# Autodesk Inventor assembly: Ensamble
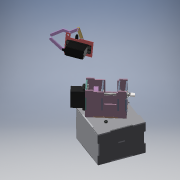
[picture p0: Inventor's stored thumbnail of the model, 180x180]
Saved by Autodesk Inventor 2019 (Build 230136000, 136)
## iProperties
Created: 2020-02-12
Part Number: Ensamble
Material: Genérico
Document SubType Name: Assembly
Designer: omar-
Author: omar-
## Documents named in this file (30)
- C:\Users\omar-\Documents\OMAR\BrazoRobotico\SERVOS\Diseño2\Ensamble.iam
- C:\Users\omar-\Documents\OMAR\BrazoRobotico\SERVOS\Diseño2\Piezas\BASE_FONDO.ipt
- C:\Users\omar-\Documents\OMAR\BrazoRobotico\SERVOS\Diseño2\Piezas\BASE_SOST.SERVO.ipt
- C:\Users\omar-\Documents\OMAR\BrazoRobotico\SERVOS\Diseño2\Servos\HS-322HD.ipt
- C:\Users\omar-\Documents\OMAR\BrazoRobotico\SERVOS\Diseño2\Piezas\BASE_TAPAFIJA.ipt
- C:\Users\omar-\Documents\OMAR\BrazoRobotico\SERVOS\Diseño2\Piezas\BASE_TAPA.ipt
- C:\Users\omar-\Documents\OMAR\BrazoRobotico\SERVOS\Diseño2\Piezas\BASE_TECHO.ipt
- C:\Users\omar-\Documents\OMAR\BrazoRobotico\SERVOS\Diseño2\Piezas\BASE_SOST.INFERIOR.ipt
- C:\Users\omar-\Documents\OMAR\BrazoRobotico\SERVOS\Diseño2\Libreria\es-ES\BS 290 SKF(12)\BS 290 SKF - SKF 6000-Z.ipt
- C:\Users\omar-\Documents\OMAR\BrazoRobotico\SERVOS\Diseño2\Piezas\BASE_PERNO.ipt
- C:\Users\omar-\Documents\OMAR\BrazoRobotico\SERVOS\Diseño2\Piezas\BASE_TUERCA.ipt
- C:\Users\omar-\Documents\OMAR\BrazoRobotico\SERVOS\Diseño2\Piezas\BASE_SOST.PERNO.ipt
- C:\Users\omar-\Documents\OMAR\BrazoRobotico\SERVOS\Diseño2\Ensamble\Design Accelerator\Conexión por perno2.iam
- C:\Users\omar-\Documents\OMAR\BrazoRobotico\SERVOS\Diseño2\Servos\SUJETADORES.ipt
- C:\Users\omar-\Documents\OMAR\BrazoRobotico\SERVOS\Diseño2\Ensamble\Design Accelerator\Conexión por perno3.iam
- C:\Users\omar-\Documents\OMAR\BrazoRobotico\SERVOS\Diseño2\Piezas\BASE_SOST.GIRATORIA.ipt
- C:\Users\omar-\Documents\OMAR\BrazoRobotico\SERVOS\Diseño2\Piezas\PINZA_SOST.SERVO.ipt
- C:\Users\omar-\Documents\OMAR\BrazoRobotico\SERVOS\Diseño2\Piezas\PINZA_UNION.ipt
- C:\Users\omar-\Documents\OMAR\BrazoRobotico\SERVOS\Diseño2\Ensamble\Design Accelerator\Conexión por perno4.iam
- C:\Users\omar-\Documents\OMAR\BrazoRobotico\SERVOS\Diseño2\Piezas\HOMBRO_SOST.EJE.ipt
- C:\Users\omar-\Documents\OMAR\BrazoRobotico\SERVOS\Diseño2\Piezas\HOMBRO_SOST.SERVO.ipt
- C:\Users\omar-\Documents\OMAR\BrazoRobotico\SERVOS\Diseño2\Servos\LKY62.ipt
- C:\Users\omar-\Documents\OMAR\BrazoRobotico\SERVOS\Diseño2\Piezas\HOMBRO_EJE.ipt
- C:\Users\omar-\Documents\OMAR\BrazoRobotico\SERVOS\Diseño2\Ensamble\Design Accelerator\Conexión por perno5.iam
- C:\Users\omar-\Documents\OMAR\BrazoRobotico\SERVOS\Diseño2\Libreria\es-ES\BS 290 SKF(29)\BS 290 SKF - SKF 626-2RS1.ipt
- C:\Users\omar-\Documents\OMAR\BrazoRobotico\SERVOS\Diseño2\Piezas\HOMBRO_SOST.COJ.ipt
- C:\Users\omar-\Documents\OMAR\BrazoRobotico\SERVOS\Diseño2\Piezas\HOMBRO_FONDO.ipt
- C:\Users\omar-\Documents\OMAR\BrazoRobotico\SERVOS\Diseño2\Piezas\HOMBRO_TAPA.LAT.ipt
- C:\Users\omar-\Documents\OMAR\BrazoRobotico\SERVOS\Diseño2\Piezas\PINZA_ESLABON.ipt
- C:\Users\omar-\Documents\OMAR\BrazoRobotico\SERVOS\Diseño2\Piezas\PINZA_DEDO.ipt
## Components (43 placed, 26 different names)
1. BASE_FONDO:1 — Coincidencia:1, Nivelación:1, Nivelación:2, Coincidencia:5, Coincidencia:8, Coincidencia:9, Nivelación:4, Coincidencia:11, Nivelación:5, Nivelación:8, Nivelación:10
2. BASE_SOST.SERVO:1 — Coincidencia:2, Coincidencia:3, Coincidencia:4, Nivelación:1, Nivelación:2, Coincidencia:10, Coincidencia:31, Coincidencia:32, Coincidencia:34
3. HS-322HD:1 — Coincidencia:2, Coincidencia:3, Coincidencia:4, Coincidencia:25
4. BASE_TAPAFIJA:1 — Coincidencia:5, Coincidencia:8, Coincidencia:9, Coincidencia:10, Nivelación:3
5. BASE_TAPAFIJA:2 — Nivelación:3, Nivelación:4, Coincidencia:11, Nivelación:6, Nivelación:7, Nivelación:9, Nivelación:12
6. BASE_TAPA:1 — Nivelación:8, Nivelación:9, Nivelación:10, Nivelación:11, Nivelación:13
7. BASE_TAPA:2 — Nivelación:5, Nivelación:6, Nivelación:7
8. BS 290 SKF- con escudo Z SKF 6000-Z:1 — Coincidencia:12, Coincidencia:18, Coincidencia:20, Coincidencia:36
9. BASE_TECHO:1 — Nivelación:11, Nivelación:12, Nivelación:13, Coincidencia:12, Coincidencia:16, Coincidencia:17, Coincidencia:23, Coincidencia:29, Coincidencia:30
10. BASE_SOST.INFERIOR:1 — Coincidencia:16, Coincidencia:17, Coincidencia:18, Coincidencia:23
11. BASE_PERNO:1 — Coincidencia:20, Coincidencia:22, Nivelación:16, Coincidencia:27, Coincidencia:35, Coincidencia:70, Coincidencia:71, Rotación:4, Rotación:5
12. BASE_TUERCA:1 — Coincidencia:22, Nivelación:16, Coincidencia:28
13. BASE_SOST.PERNO:1 — Coincidencia:24, Coincidencia:26, Coincidencia:28, Rotación:4
14. BASE_SOST.PERNO:2 — Coincidencia:24, Coincidencia:25, Coincidencia:26, Coincidencia:27
15. Conexión por perno:1 [sub-assembly] — Coincidencia:29, Coincidencia:30
16. SUJETADORES:1 — Coincidencia:31, Coincidencia:32, Coincidencia:33
17. Conexión por perno:2 [sub-assembly] — Coincidencia:33, Coincidencia:34
18. BASE_SOST.GIRATORIA:1 — Coincidencia:35, Coincidencia:36, Coincidencia:72
19. PINZA_SOST.SERVO:1 — Coincidencia:37, Coincidencia:38, Coincidencia:39, Coincidencia:41, Nivelación:18, Coincidencia:43, Coincidencia:69, Coincidencia:77, Coincidencia:80
20. HS-322HD:2 — Coincidencia:37, Coincidencia:38, Coincidencia:39, Nivelación:17, Coincidencia:40
21. PINZA_UNION:1 — Nivelación:17, Coincidencia:40, Coincidencia:73, Coincidencia:74, Coincidencia:75, Coincidencia:76
22. SUJETADORES:2 — Coincidencia:41, Nivelación:18, Coincidencia:42
23. Conexión por perno:3 [sub-assembly] — Coincidencia:42, Coincidencia:43, Coincidencia:69
24. HOMBRO_SOST.EJE:1 — Coincidencia:44, Coincidencia:45, Coincidencia:52, Coincidencia:53, Nivelación:19
25. HOMBRO_SOST.SERVO:1 — Coincidencia:46, Coincidencia:47, Coincidencia:48, Nivelación:20, Nivelación:21, Coincidencia:62, Coincidencia:68, Nivelación:24, Nivelación:27, Nivelación:28, Nivelación:29
26. LKY62:1 — Coincidencia:44, Coincidencia:45, Coincidencia:46, Coincidencia:47, Coincidencia:48, Coincidencia:49, Coincidencia:50, Coincidencia:56
27. Conexión por perno:4 [sub-assembly] — Coincidencia:49, Coincidencia:50, Coincidencia:68
28. HOMBRO_SOST.EJE:2 — Coincidencia:54, Coincidencia:55, Rotación:2
29. HOMBRO_SOST.EJE:3 — Coincidencia:52, Coincidencia:53, Coincidencia:54, Coincidencia:55
30. BS 290 SKF- con dos juntas RS1 SKF 626-2RS1:1 — Coincidencia:59, Coincidencia:66
31. BS 290 SKF- con dos juntas RS1 SKF 626-2RS1:2 — Coincidencia:58, Coincidencia:64
32. BS 290 SKF- con dos juntas RS1 SKF 626-2RS1:3 — Coincidencia:57, Nivelación:22
33. HOMBRO_EJE:1 — Coincidencia:56, Coincidencia:57, Coincidencia:58, Coincidencia:59, Rotación:2, Nivelación:19, Coincidencia:60, Coincidencia:61, Coincidencia:65, Coincidencia:66
34. HOMBRO_SOST.COJ:1 — Coincidencia:60, Nivelación:20, Nivelación:22, Coincidencia:62, Coincidencia:63
35. HOMBRO_SOST.COJ:2 — Coincidencia:61, Nivelación:21, Coincidencia:63, Coincidencia:64, Nivelación:23, Coincidencia:67, Nivelación:26, Nivelación:30
36. HOMBRO_SOST.COJ:3 — Coincidencia:65, Nivelación:23, Coincidencia:67, Nivelación:25, Nivelación:31, Nivelación:32
37. HOMBRO_FONDO:1 — Nivelación:24, Nivelación:25, Nivelación:26, Coincidencia:70, Coincidencia:71, Coincidencia:72, Rotación:5
38. HOMBRO_TAPA.LAT:2 — Nivelación:30, Nivelación:31, Nivelación:32
39. PINZA_ESLABON:1 — Coincidencia:73, Coincidencia:75, Coincidencia:81, Coincidencia:82
40. PINZA_ESLABON:2 — Coincidencia:74, Coincidencia:76, Coincidencia:78, Coincidencia:79
41. PINZA_DEDO:1 — Coincidencia:77, Coincidencia:78, Coincidencia:79
42. PINZA_DEDO:2 — Coincidencia:80, Coincidencia:81, Coincidencia:82
43. HOMBRO_TAPA.LAT:1 — Nivelación:27, Nivelación:28, Nivelación:29
## Relationships (107: Mate 74, Flush 30, RelateRotation 3)
- Coincidencia:1 [Mate]: BASE_FONDO:1
- Coincidencia:2 [Mate]: BASE_SOST.SERVO:1 ↔ HS-322HD:1
- Coincidencia:3 [Mate]: BASE_SOST.SERVO:1 ↔ HS-322HD:1
- Coincidencia:4 [Mate] (1 mm): BASE_SOST.SERVO:1 ↔ HS-322HD:1
- Nivelación:1 [Flush]: BASE_FONDO:1 ↔ BASE_SOST.SERVO:1
- Nivelación:2 [Flush] (35 mm): BASE_FONDO:1 ↔ BASE_SOST.SERVO:1
- Coincidencia:5 [Mate]: BASE_FONDO:1 ↔ BASE_TAPAFIJA:1
- Coincidencia:8 [Mate]: BASE_FONDO:1 ↔ BASE_TAPAFIJA:1
- Coincidencia:9 [Mate]: BASE_FONDO:1 ↔ BASE_TAPAFIJA:1
- Coincidencia:10 [Mate]: BASE_SOST.SERVO:1 ↔ BASE_TAPAFIJA:1
- Nivelación:3 [Flush]: BASE_TAPAFIJA:1 ↔ BASE_TAPAFIJA:2
- Nivelación:4 [Flush]: BASE_FONDO:1 ↔ BASE_TAPAFIJA:2
- Coincidencia:11 [Mate]: BASE_FONDO:1 ↔ BASE_TAPAFIJA:2
- Nivelación:5 [Flush]: BASE_FONDO:1 ↔ BASE_TAPA:2
- Nivelación:6 [Flush]: BASE_TAPAFIJA:2 ↔ BASE_TAPA:2
- Nivelación:7 [Flush]: BASE_TAPAFIJA:2 ↔ BASE_TAPA:2
- Nivelación:8 [Flush]: BASE_FONDO:1 ↔ BASE_TAPA:1
- Nivelación:9 [Flush]: BASE_TAPAFIJA:2 ↔ BASE_TAPA:1
- Nivelación:10 [Flush]: BASE_FONDO:1 ↔ BASE_TAPA:1
- Nivelación:11 [Flush]: BASE_TAPA:1 ↔ BASE_TECHO:1
- Nivelación:12 [Flush]: BASE_TAPAFIJA:2 ↔ BASE_TECHO:1
- Nivelación:13 [Flush]: BASE_TAPA:1 ↔ BASE_TECHO:1
- Coincidencia:12 [Mate]: BS 290 SKF- con escudo Z SKF 6000-Z:1 ↔ BASE_TECHO:1
- Coincidencia:16 [Mate]: BASE_TECHO:1 ↔ BASE_SOST.INFERIOR:1
- Coincidencia:17 [Mate]: BASE_TECHO:1 ↔ BASE_SOST.INFERIOR:1
- Coincidencia:18 [Mate]: BS 290 SKF- con escudo Z SKF 6000-Z:1 ↔ BASE_SOST.INFERIOR:1
- Coincidencia:20 [Mate]: BS 290 SKF- con escudo Z SKF 6000-Z:1 ↔ BASE_PERNO:1
- Coincidencia:22 [Mate]: BASE_PERNO:1 ↔ BASE_TUERCA:1
- Nivelación:16 [Flush]: BASE_PERNO:1 ↔ BASE_TUERCA:1
- Coincidencia:23 [Mate]: BASE_TECHO:1 ↔ BASE_SOST.INFERIOR:1
- Coincidencia:24 [Mate]: BASE_SOST.PERNO:1 ↔ BASE_SOST.PERNO:2
- Coincidencia:25 [Mate]: HS-322HD:1 ↔ BASE_SOST.PERNO:2
- Coincidencia:26 [Mate]: BASE_SOST.PERNO:1 ↔ BASE_SOST.PERNO:2
- Coincidencia:27 [Mate]: BASE_PERNO:1 ↔ BASE_SOST.PERNO:2
- Coincidencia:28 [Mate]: BASE_TUERCA:1 ↔ BASE_SOST.PERNO:1
- Coincidencia:29 [Mate]: BASE_TECHO:1 ↔ Conexión por perno:1
- Coincidencia:30 [Mate]: BASE_TECHO:1 ↔ Conexión por perno:1
- Coincidencia:31 [Mate]: BASE_SOST.SERVO:1 ↔ SUJETADORES:1
- Coincidencia:32 [Mate] (3.5 mm): BASE_SOST.SERVO:1 ↔ SUJETADORES:1
- Coincidencia:33 [Mate]: SUJETADORES:1 ↔ Conexión por perno:2
- Coincidencia:34 [Mate]: BASE_SOST.SERVO:1 ↔ Conexión por perno:2
- Coincidencia:35 [Mate]: BASE_PERNO:1 ↔ BASE_SOST.GIRATORIA:1
- Coincidencia:36 [Mate]: BS 290 SKF- con escudo Z SKF 6000-Z:1 ↔ BASE_SOST.GIRATORIA:1
- Coincidencia:37 [Mate] (1 mm): PINZA_SOST.SERVO:1 ↔ HS-322HD:2
- Coincidencia:38 [Mate]: PINZA_SOST.SERVO:1 ↔ HS-322HD:2
- Coincidencia:39 [Mate]: PINZA_SOST.SERVO:1 ↔ HS-322HD:2
- Nivelación:17 [Flush] (-0.1 mm): HS-322HD:2 ↔ PINZA_UNION:1
- Coincidencia:40 [Mate]: HS-322HD:2 ↔ PINZA_UNION:1
- Coincidencia:41 [Mate]: PINZA_SOST.SERVO:1 ↔ SUJETADORES:2
- Nivelación:18 [Flush] (3.5 mm): PINZA_SOST.SERVO:1 ↔ SUJETADORES:2
- Coincidencia:42 [Mate]: SUJETADORES:2 ↔ Conexión por perno:3
- Coincidencia:43 [Mate]: PINZA_SOST.SERVO:1 ↔ Conexión por perno:3
- Coincidencia:44 [Mate]: HOMBRO_SOST.EJE:1 ↔ LKY62:1
- Coincidencia:45 [Mate] (8.18 mm): HOMBRO_SOST.EJE:1 ↔ LKY62:1
- Coincidencia:46 [Mate] (1 mm): HOMBRO_SOST.SERVO:1 ↔ LKY62:1
- Coincidencia:47 [Mate]: HOMBRO_SOST.SERVO:1 ↔ LKY62:1
- Coincidencia:48 [Mate]: HOMBRO_SOST.SERVO:1 ↔ LKY62:1
- Coincidencia:49 [Mate]: LKY62:1 ↔ Conexión por perno:4
- Coincidencia:50 [Mate]: LKY62:1 ↔ Conexión por perno:4
- Coincidencia:52 [Mate]: HOMBRO_SOST.EJE:1 ↔ HOMBRO_SOST.EJE:3
- Coincidencia:53 [Mate]: HOMBRO_SOST.EJE:1 ↔ HOMBRO_SOST.EJE:3
- Coincidencia:54 [Mate]: HOMBRO_SOST.EJE:2 ↔ HOMBRO_SOST.EJE:3
- Coincidencia:55 [Mate]: HOMBRO_SOST.EJE:2 ↔ HOMBRO_SOST.EJE:3
- Coincidencia:56 [Mate]: LKY62:1 ↔ HOMBRO_EJE:1
- Coincidencia:57 [Mate]: BS 290 SKF- con dos juntas RS1 SKF 626-2RS1:3 ↔ HOMBRO_EJE:1
- Coincidencia:58 [Mate]: BS 290 SKF- con dos juntas RS1 SKF 626-2RS1:2 ↔ HOMBRO_EJE:1
- Coincidencia:59 [Mate]: BS 290 SKF- con dos juntas RS1 SKF 626-2RS1:1 ↔ HOMBRO_EJE:1
- Rotación:2 [RelateRotation] (1 ul): HOMBRO_SOST.EJE:2 ↔ HOMBRO_EJE:1
- Nivelación:19 [Flush]: HOMBRO_SOST.EJE:1 ↔ HOMBRO_EJE:1
- Coincidencia:60 [Mate]: HOMBRO_EJE:1 ↔ HOMBRO_SOST.COJ:1
- Nivelación:20 [Flush]: HOMBRO_SOST.SERVO:1 ↔ HOMBRO_SOST.COJ:1
- Coincidencia:61 [Mate]: HOMBRO_EJE:1 ↔ HOMBRO_SOST.COJ:2
- Nivelación:21 [Flush]: HOMBRO_SOST.SERVO:1 ↔ HOMBRO_SOST.COJ:2
- Nivelación:22 [Flush] (-1 mm): BS 290 SKF- con dos juntas RS1 SKF 626-2RS1:3 ↔ HOMBRO_SOST.COJ:1
- Coincidencia:62 [Mate] (30 mm): HOMBRO_SOST.SERVO:1 ↔ HOMBRO_SOST.COJ:1
- Coincidencia:63 [Mate] (30 mm): HOMBRO_SOST.COJ:1 ↔ HOMBRO_SOST.COJ:2
- Coincidencia:64 [Mate] (1 mm): BS 290 SKF- con dos juntas RS1 SKF 626-2RS1:2 ↔ HOMBRO_SOST.COJ:2
- Coincidencia:65 [Mate]: HOMBRO_EJE:1 ↔ HOMBRO_SOST.COJ:3
- Nivelación:23 [Flush]: HOMBRO_SOST.COJ:2 ↔ HOMBRO_SOST.COJ:3
- Coincidencia:66 [Mate] (1 mm): BS 290 SKF- con dos juntas RS1 SKF 626-2RS1:1 ↔ HOMBRO_EJE:1
- Coincidencia:67 [Mate] (12 mm): HOMBRO_SOST.COJ:2 ↔ HOMBRO_SOST.COJ:3
- Coincidencia:68 [Mate]: HOMBRO_SOST.SERVO:1 ↔ Conexión por perno:4
- Coincidencia:69 [Mate]: PINZA_SOST.SERVO:1 ↔ Conexión por perno:3
- Nivelación:24 [Flush]: HOMBRO_SOST.SERVO:1 ↔ HOMBRO_FONDO:1
- Nivelación:25 [Flush]: HOMBRO_SOST.COJ:3 ↔ HOMBRO_FONDO:1
- Nivelación:26 [Flush]: HOMBRO_SOST.COJ:2 ↔ HOMBRO_FONDO:1
- Nivelación:27 [Flush]: HOMBRO_SOST.SERVO:1 ↔ HOMBRO_TAPA.LAT:1
- Nivelación:28 [Flush]: HOMBRO_SOST.SERVO:1 ↔ HOMBRO_TAPA.LAT:1
- Nivelación:29 [Flush]: HOMBRO_SOST.SERVO:1 ↔ HOMBRO_TAPA.LAT:1
- Nivelación:30 [Flush]: HOMBRO_SOST.COJ:2 ↔ HOMBRO_TAPA.LAT:2
- Nivelación:31 [Flush]: HOMBRO_SOST.COJ:3 ↔ HOMBRO_TAPA.LAT:2
- Nivelación:32 [Flush]: HOMBRO_SOST.COJ:3 ↔ HOMBRO_TAPA.LAT:2
- Coincidencia:70 [Mate]: BASE_PERNO:1 ↔ HOMBRO_FONDO:1
- Coincidencia:71 [Mate]: BASE_PERNO:1 ↔ HOMBRO_FONDO:1
- Coincidencia:72 [Mate]: BASE_SOST.GIRATORIA:1 ↔ HOMBRO_FONDO:1
- Rotación:4 [RelateRotation] (1 ul): BASE_PERNO:1 ↔ BASE_SOST.PERNO:1
- Rotación:5 [RelateRotation] (1 ul): BASE_PERNO:1 ↔ HOMBRO_FONDO:1
- Coincidencia:73 [Mate]: PINZA_UNION:1 ↔ PINZA_ESLABON:1
- Coincidencia:74 [Mate]: PINZA_UNION:1 ↔ PINZA_ESLABON:2
- Coincidencia:75 [Mate]: PINZA_UNION:1 ↔ PINZA_ESLABON:1
- Coincidencia:76 [Mate]: PINZA_UNION:1 ↔ PINZA_ESLABON:2
- Coincidencia:77 [Mate]: PINZA_SOST.SERVO:1 ↔ PINZA_DEDO:1
- Coincidencia:78 [Mate]: PINZA_ESLABON:2 ↔ PINZA_DEDO:1
- Coincidencia:79 [Mate]: PINZA_ESLABON:2 ↔ PINZA_DEDO:1
- Coincidencia:80 [Mate]: PINZA_SOST.SERVO:1 ↔ PINZA_DEDO:2
- Coincidencia:81 [Mate]: PINZA_ESLABON:1 ↔ PINZA_DEDO:2
- Coincidencia:82 [Mate]: PINZA_ESLABON:1 ↔ PINZA_DEDO:2
